# Autodesk Inventor assembly: 後ウイング1_MIR
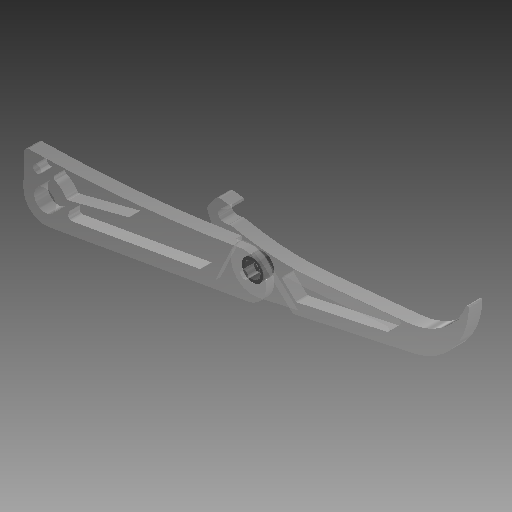
[picture p0: Inventor's stored thumbnail of the model, 512x512]
Saved by Autodesk Inventor 2020 (Build 240168000, 168)
## iProperties
Created: 2019-09-05
Part Number: 後ウイング1_MIR
Document SubType Name: Assembly
Designer: 雪村
Mass: 12.1457 g
Surface Area: 91.6324 cm^2
Volume: 10.1049 cm^3
Density: 1.20196 g/cm^3
Author: 雪村
## Documents named in this file (4)
- C:\Users\white\Documents\SRDC\SRDC\Inventor_2017\2018年機体\2020年4年機体\後ウイング1_MIR.iam
- C:\Users\white\Documents\SRDC\SRDC\Inventor_2017\2018年機体\2020年4年機体\後ウイング1.1_MIR.ipt
- C:\Users\white\Documents\SRDC\SRDC\Inventor_2017\2018年機体\2020年4年機体\後ウイング1.2_MIR.ipt
- C:\Users\white\Documents\SRDC\SRDC\Inventor_2017\2018年機体\パーツ\オイレス060804.ipt
## Components (3 placed, 3 different names)
1. 後ウイング1.1_MIR:1 — 挿入:1
2. 後ウイング1.2_MIR:1 — 挿入:2
3. オイレス060804:1 — 挿入:2, 挿入:1
## Relationships (2: Insert 2)
- 挿入:2 [Insert]: 後ウイング1.2_MIR:1 ↔ オイレス060804:1
- 挿入:1 [Insert]: 後ウイング1.1_MIR:1 ↔ オイレス060804:1
